# Autodesk Inventor assembly: Ballshifter Cylinder
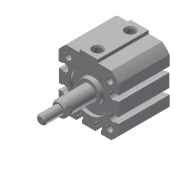
[picture p0: Inventor's stored thumbnail of the model, 180x180]
Saved by Autodesk Inventor 2013 (Build 170138000, 138)
## iProperties
Created: 2013-04-08
Part Number: Ballshifter Cylinder
Document SubType Name: Assembly
Designer: Niemitalo_Dan
Author: Niemitalo_Dan
## Documents named in this file (3)
- \\lmss\students\Robotics\CAD Files\COTS Parts\Gearboxes\Components\VexPro Ballshifter Components\Ballshifter Cylinder.iam
- \\lmss\students\Robotics\CAD Files\COTS Parts\Gearboxes\Components\VexPro Ballshifter Components\Ballshifter Cylinder Body.ipt
- \\lmss\students\Robotics\CAD Files\COTS Parts\Gearboxes\Components\VexPro Ballshifter Components\Ballshifter Cylinder Rod.ipt
## Components (2 placed, 2 different names)
1. Ballshifter Cylinder Body:1 — Mate:1, Flush:1, Angle:1
2. Ballshifter Cylinder Rod:1 — Mate:1, Flush:1, Angle:1
## Relationships (3: Mate 1, Flush 1, Angle 1)
- Mate:1: Ballshifter Cylinder Body:1 ↔ Ballshifter Cylinder Rod:1
- Flush:1 (3.175 mm): Ballshifter Cylinder Body:1 ↔ Ballshifter Cylinder Rod:1
- Angle:1 (0 deg): Ballshifter Cylinder Body:1 ↔ Ballshifter Cylinder Rod:1
